# Autodesk Inventor assembly: Assembly Senstable
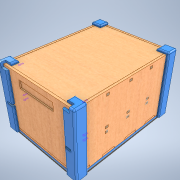
[picture p0: Inventor's stored thumbnail of the model, 180x180]
Saved by Autodesk Inventor 2021 (Build 250183000, 183)
## iProperties
Created: 2021-03-11
Part Number: Assembly Senstable
Document SubType Name: Assembly
Designer: ZiweZhang
Author: ZiweZhang
## Documents named in this file (13)
- Z:\ziwez\Documents\GitHub\SensTable2\Design\Versie 2\Inventor\SensorDoosje\Assembly Senstable.iam
- Assembly SensorDoosje.iam
- Z:\ziwez\Documents\GitHub\SensTable2\Design\Versie 2\Inventor\SensorDoosje\DoosjeOnderkant.ipt
- Z:\ziwez\Documents\GitHub\SensTable2\Design\Versie 2\Inventor\SensorDoosje\DoosjeVoorkant.ipt
- Z:\ziwez\Documents\GitHub\SensTable2\Design\Versie 2\Inventor\SensorDoosje\DoosjeRechter-Linkerkant.ipt
- Z:\ziwez\Documents\GitHub\SensTable2\Design\Versie 2\Inventor\SensorDoosje\DoosjeHoeken.ipt
- Z:\ziwez\Documents\GitHub\SensTable2\Design\Versie 2\Inventor\SensorDoosje\DoosjeGrid.ipt
- Z:\ziwez\Documents\GitHub\SensTable2\Design\Versie 2\Inventor\SensorDoosje\steun.ipt
- Z:\ziwez\Documents\GitHub\SensTable2\Design\Versie 2\Inventor\SensorDoosje\DoosjeHoekenVoorLinks.ipt
- Z:\ziwez\Documents\GitHub\SensTable2\Design\Versie 2\Inventor\SensorDoosje\DoosjeAchterkant.ipt
- Z:\ziwez\Documents\GitHub\SensTable2\Design\Versie 2\Inventor\SensorDoosje\DoosjeHoekenVoorRechts.ipt
- Z:\ziwez\Documents\GitHub\SensTable2\Design\Versie 2\Inventor\SensorDoosje\DoosjeBovenkant.ipt
- D:\School\Projecten\Project 78 - Senstable\Design\Versie 2\Inventor\SensorDoosje\Grid.ipt
## Components (18 placed, 9 different names)
1. DoosjeBovenkant:1 — Rigid:23
2. DoosjeOnderkant:1 — Rigid:22, Rigid:25
3. DoosjeAchterkant:1 — Rigid:9, Rigid:19, Rigid:20, Rigid:21
4. DoosjeVoorkant:2 — Rigid:24
5. DoosjeRechter-Linkerkant:1 — Rigid:13, Rigid:14, Rigid:15, Rigid:17, Rigid:21
6. DoosjeRechter-Linkerkant:2 — Rigid:9, Rigid:10, Rigid:11, Rigid:12, Rigid:18, Rigid:22, Rigid:24
7. DoosjeGrid:1 — Rigid:25
8. DoosjeHoeken:1 — Rigid:20
9. DoosjeHoeken:2 — Rigid:19
10. DoosjeHoeken:3 — Rigid:17
11. DoosjeHoeken:4 — Rigid:18
12. steun:1 — Rigid:14
13. steun:2 — Rigid:12
14. steun:3 — Rigid:15
15. steun:4 — Rigid:11
16. steun:5 — Rigid:10
17. steun:6 — Rigid:13, Rigid:23
18. Grid:1
## Relationships (16: WeldJoint 16)
- Rigid:9 [WeldJoint]: DoosjeAchterkant:1 ↔ DoosjeRechter-Linkerkant:2
- Rigid:10 [WeldJoint]: DoosjeRechter-Linkerkant:2 ↔ steun:5
- Rigid:11 [WeldJoint]: DoosjeRechter-Linkerkant:2 ↔ steun:4
- Rigid:12 [WeldJoint]: DoosjeRechter-Linkerkant:2 ↔ steun:2
- Rigid:13 [WeldJoint]: DoosjeRechter-Linkerkant:1 ↔ steun:6
- Rigid:14 [WeldJoint]: DoosjeRechter-Linkerkant:1 ↔ steun:1
- Rigid:15 [WeldJoint]: DoosjeRechter-Linkerkant:1 ↔ steun:3
- Rigid:17 [WeldJoint]: DoosjeRechter-Linkerkant:1 ↔ DoosjeHoeken:3
- Rigid:18 [WeldJoint]: DoosjeRechter-Linkerkant:2 ↔ DoosjeHoeken:4
- Rigid:19 [WeldJoint]: DoosjeAchterkant:1 ↔ DoosjeHoeken:2
- Rigid:20 [WeldJoint]: DoosjeAchterkant:1 ↔ DoosjeHoeken:1
- Rigid:21 [WeldJoint]: DoosjeAchterkant:1 ↔ DoosjeRechter-Linkerkant:1
- Rigid:22 [WeldJoint]: DoosjeOnderkant:1 ↔ DoosjeRechter-Linkerkant:2
- Rigid:23 [WeldJoint]: DoosjeBovenkant:1 ↔ steun:6
- Rigid:24 [WeldJoint]: DoosjeVoorkant:2 ↔ DoosjeRechter-Linkerkant:2
- Rigid:25 [WeldJoint]: DoosjeOnderkant:1 ↔ DoosjeGrid:1
